# Autodesk Inventor assembly: DISH antenna assembly
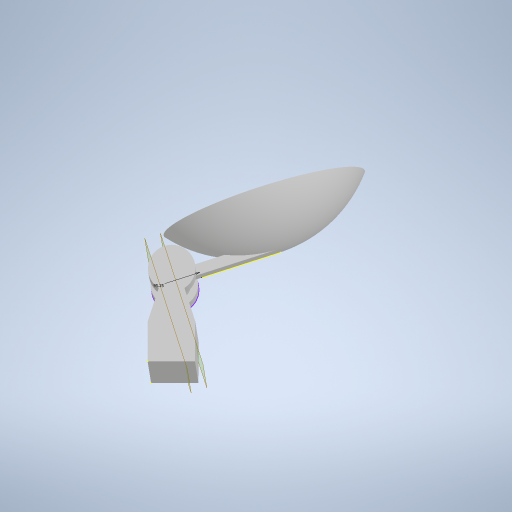
[picture p0: Inventor's stored thumbnail of the model, 512x512]
Saved by Autodesk Inventor 2024 (Build 280153000, 153)
## iProperties
Created: 2023-07-01
Part Number: DISH antenna assembly
Document SubType Name: Assembly
Designer: hp
Author: hp
## Documents named in this file (3)
- D:\EG\DISH antenna assembly.iam
- C:\Users\hp\Desktop\Dish antenna base.ipt
- D:\EG\Dish final.ipt
## Components (2 placed, 2 different names)
1. Dish antenna base:1 — Mate:1, Mate:2, Mate:3
2. Dish final:1 — Mate:1, Mate:2, Mate:3
## Relationships (3: Mate 3)
- Mate:1: Dish antenna base:1 ↔ Dish final:1
- Mate:2: Dish antenna base:1 ↔ Dish final:1
- Mate:3: Dish antenna base:1 ↔ Dish final:1
